# Autodesk Inventor assembly: Configuration 1
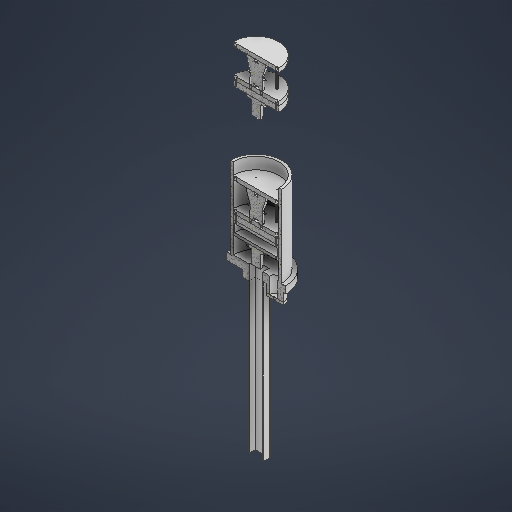
[picture p0: Inventor's stored thumbnail of the model, 512x512]
Saved by Autodesk Inventor 2025 (Build 290162000, 162)
## iProperties
Created: 2024-06-05
Part Number: Configuration 1
Document SubType Name: Assembly
Designer: AdminForWorker
Title: Printer Assembly v13
Author: AdminForWorker
## Documents named in this file (23)
- C:\Users\mayhe\OneDrive\Documents\GitHub\In-situ-monitoring-of-powder-bed-fusion-additive-manufacturing\system_development\Orichalcum\v0.2\Hardware_design\Full Printer Assembly\Printer Assembly.iam
- C:\Users\mayhe\OneDrive\Documents\GitHub\In-situ-monitoring-of-powder-bed-fusion-additive-manufacturing\system_development\Orichalcum\v0.2\Hardware_design\Full Printer Assembly\Printer Body v6.ipt
- C:\Users\mayhe\OneDrive\Documents\GitHub\In-situ-monitoring-of-powder-bed-fusion-additive-manufacturing\system_development\Orichalcum\v0.2\Hardware_design\Full Printer Assembly\Printer Frame.ipt
- C:\Users\mayhe\OneDrive\Documents\GitHub\In-situ-monitoring-of-powder-bed-fusion-additive-manufacturing\system_development\Orichalcum\v0.2\Hardware_design\Full Printer Assembly\overhead laser unit v1.ipt
- C:\Users\mayhe\OneDrive\Documents\GitHub\In-situ-monitoring-of-powder-bed-fusion-additive-manufacturing\system_development\Orichalcum\v0.2\Hardware_design\Full Printer Assembly\Part4.ipt
- C:\Users\mayhe\OneDrive\Documents\GitHub\In-situ-monitoring-of-powder-bed-fusion-additive-manufacturing\system_development\Orichalcum\v0.2\Hardware_design\custom-cover\cover\Updated Cover.ipt
- C:\Users\mayhe\OneDrive\Documents\GitHub\In-situ-monitoring-of-powder-bed-fusion-additive-manufacturing\system_development\Orichalcum\v0.2\Hardware_design\custom-cover\cylinder-parts\final-parts\Cylinder Bottom Ring.ipt
- C:\Users\mayhe\OneDrive\Documents\GitHub\In-situ-monitoring-of-powder-bed-fusion-additive-manufacturing\system_development\Orichalcum\v0.2\Hardware_design\custom-cover\cylinder-parts\final-parts\Cylinder Slidey Bit Housing.ipt
- C:\Users\mayhe\OneDrive\Documents\GitHub\In-situ-monitoring-of-powder-bed-fusion-additive-manufacturing\system_development\Orichalcum\v0.2\Hardware_design\custom-cover\cylinder-parts\Cylinder 80-20 Spacer_1.ipt
- C:\Users\mayhe\OneDrive\Documents\GitHub\In-situ-monitoring-of-powder-bed-fusion-additive-manufacturing\system_development\Orichalcum\v0.2\Hardware_design\custom-cover\cylinder-parts\Cylinder 80-20 Spacer_2.ipt
- C:\Users\mayhe\OneDrive\Documents\GitHub\In-situ-monitoring-of-powder-bed-fusion-additive-manufacturing\system_development\Orichalcum\v0.2\Hardware_design\custom-cover\8020-parts\20-2020-300.ipt
- C:\Users\mayhe\OneDrive\Documents\GitHub\In-situ-monitoring-of-powder-bed-fusion-additive-manufacturing\system_development\Orichalcum\v0.2\Hardware_design\custom-cover\cylinder-parts\cylinder-segments\Cylinder Segment .ipt
- C:\Users\mayhe\OneDrive\Documents\GitHub\In-situ-monitoring-of-powder-bed-fusion-additive-manufacturing\system_development\Orichalcum\v0.2\Hardware_design\custom-cover\cylinder-parts\final-parts\Cylinder Segment - 01.ipt
- C:\Users\mayhe\OneDrive\Documents\GitHub\In-situ-monitoring-of-powder-bed-fusion-additive-manufacturing\system_development\Orichalcum\v0.2\Hardware_design\custom-cover\cylinder-parts\final-parts\Cylinder Segment - Face.ipt
- C:\Users\mayhe\OneDrive\Documents\GitHub\In-situ-monitoring-of-powder-bed-fusion-additive-manufacturing\system_development\Orichalcum\v0.2\Hardware_design\custom-cover\cylinder-parts\final-parts\Cylinder Segment - 09.ipt
- C:\Users\mayhe\OneDrive\Documents\GitHub\In-situ-monitoring-of-powder-bed-fusion-additive-manufacturing\system_development\Orichalcum\v0.2\Hardware_design\custom-cover\cylinder-parts\final-parts\Cylinder Segment - 10.ipt
- C:\Users\mayhe\OneDrive\Documents\GitHub\In-situ-monitoring-of-powder-bed-fusion-additive-manufacturing\system_development\Orichalcum\v0.2\Hardware_design\custom-cover\cylinder-parts\cylinder-segments\Head Thing.ipt
- C:\Users\mayhe\OneDrive\Documents\GitHub\In-situ-monitoring-of-powder-bed-fusion-additive-manufacturing\system_development\Orichalcum\v0.2\Hardware_design\Full Printer Assembly\Plunger.ipt
- C:\Users\mayhe\OneDrive\Documents\GitHub\In-situ-monitoring-of-powder-bed-fusion-additive-manufacturing\system_development\Orichalcum\v0.2\Hardware_design\pzt-parts\PZT Assembly.iam
- C:\Users\mayhe\OneDrive\Documents\GitHub\In-situ-monitoring-of-powder-bed-fusion-additive-manufacturing\system_development\Orichalcum\v0.2\Hardware_design\Full Printer Assembly\Adapter Plate.ipt
- C:\Users\mayhe\OneDrive\Documents\GitHub\In-situ-monitoring-of-powder-bed-fusion-additive-manufacturing\system_development\Orichalcum\v0.2\Hardware_design\Full Printer Assembly\Build Plate.ipt
- C:\Users\mayhe\OneDrive\Documents\GitHub\In-situ-monitoring-of-powder-bed-fusion-additive-manufacturing\system_development\Orichalcum\v0.2\Hardware_design\Full Printer Assembly\Bottom Cap outlet.ipt
- C:\Users\mayhe\OneDrive\Documents\GitHub\In-situ-monitoring-of-powder-bed-fusion-additive-manufacturing\system_development\Orichalcum\v0.2\Hardware_design\pzt-parts\Capsule.ipt
## Components (28 placed, 21 different names)
1. Printer Frame:1 — Flush:1, Mate:1, Mate:2, Mate:3, Flush:2, Flush:3, Rotational:5, Rotational:6, Angle:3, Angle:4
2. Printer Body v6:1 — Flush:1, Mate:1, Mate:2, Mate:5, Mate:6, Mate:7, Angle:2
3. overhead laser unit v1:1 — Mate:4, Angle:1, Flush:4
4. Part4:1 — Mate:3, Flush:2, Flush:3, Mate:4, Angle:1, Flush:4
5. Plunger:1 — Rotational:6
6. Plunger:2 — Rotational:5, Cylindrical:1, Rotational:9, Mate:68, Angle:2, Cylindrical:2
7. Bottom Cap outlet:1 — Rotational:9, Mate:68
8. Updated Cover:1 — Mate:5, Mate:6, Mate:7, Rotational:4, Mate:53
9. Cylinder 80-20 Spacer_1:2 — Flush:5, Mate:29, Flush:6, Mate:30, Mate:59
10. Cylinder 80-20 Spacer_2:1 — Mate:26, Mate:60, Mate:61, Mate:62
11. Cylinder 80-20 Spacer_2:2 — Mate:47, Mate:54, Mate:55, Mate:56, Flush:7, Mate:57
12. Cylinder 80-20 Spacer_1:3 — Mate:64, Mate:65, Mate:66
13. 20-2020-300:1 — Mate:29, Flush:6, Mate:56, Flush:7, Mate:58
14. 20-2020-300:2 — Mate:26, Flush:5, Mate:52, Mate:63
15. Cylinder Segment - 01:1 — Mate:30, Mate:47, Rotational:2, Mate:48
16. Cylinder Slidey Bit Housing:1 — Rotational:2, Mate:48, Mate:50, Mate:51
17. Cylinder Segment - Face:2 — Rotational:3
18. Cylinder Segment - 09:3 — Mate:51, Mate:52
19. Cylinder Segment - 10:4 — Mate:50
20. Head Thing:1 — Rotational:3
21. Cylinder Bottom Ring:1 — Rotational:4, Mate:53, Mate:54, Mate:55, Mate:57, Mate:58, Mate:59, Mate:60, Mate:61, Mate:62, Mate:63, Mate:64, Mate:65, Mate:66
22. Build Plate:1 — Rotational:7, Rotational:8, Mate:67
23. Adapter Plate:1 — Rotational:7
24. PZT Assembly:1 [sub-assembly] — Rotational:8, Mate:67, Cylindrical:1, Angle:3
25. Capsule:1 — Rotational:10, Rotational:12, Mate:70
26. PZT Assembly:3 [sub-assembly] — Rotational:11, Cylindrical:2, Angle:4, Mate:69
27. Build Plate:3 — Rotational:10, Rotational:11, Mate:69, Mate:70
28. Adapter Plate:2 — Rotational:12
## Relationships (57: Mate 33, RevoluteJoint 11, Flush 7, Angle 4, CylindricalJoint 2)
- Flush:1: Printer Frame:1 ↔ Printer Body v6:1
- Mate:1: Printer Frame:1 ↔ Printer Body v6:1
- Mate:2 (92.5 mm): Printer Frame:1 ↔ Printer Body v6:1
- Mate:3: Printer Frame:1 ↔ Part4:1
- Flush:2 (28.5 mm): Printer Frame:1 ↔ Part4:1
- Flush:3 (-27 mm): Printer Frame:1 ↔ Part4:1
- Mate:4: overhead laser unit v1:1 ↔ Part4:1
- Angle:1 (179.9998 deg): overhead laser unit v1:1 ↔ Part4:1
- Flush:4 (-30 mm): overhead laser unit v1:1 ↔ Part4:1
- Mate:5: Printer Body v6:1 ↔ Updated Cover:1
- Mate:6: Printer Body v6:1 ↔ Updated Cover:1
- Mate:7: Printer Body v6:1 ↔ Updated Cover:1
- Mate:26: Cylinder 80-20 Spacer_2:1 ↔ 20-2020-300:2
- Flush:5: Cylinder 80-20 Spacer_1:2 ↔ 20-2020-300:2
- Mate:29: Cylinder 80-20 Spacer_1:2 ↔ 20-2020-300:1
- Flush:6: Cylinder 80-20 Spacer_1:2 ↔ 20-2020-300:1
- Mate:30: Cylinder 80-20 Spacer_1:2 ↔ Cylinder Segment - 01:1
- Mate:47: Cylinder 80-20 Spacer_2:2 ↔ Cylinder Segment - 01:1
- Rotational:2 [RevoluteJoint]: Cylinder Segment - 01:1 ↔ Cylinder Slidey Bit Housing:1
- Mate:48: Cylinder Segment - 01:1 ↔ Cylinder Slidey Bit Housing:1
- Mate:50: Cylinder Slidey Bit Housing:1 ↔ Cylinder Segment - 10:4
- Mate:51: Cylinder Slidey Bit Housing:1 ↔ Cylinder Segment - 09:3
- Mate:52: 20-2020-300:2 ↔ Cylinder Segment - 09:3
- Rotational:3 [RevoluteJoint]: Cylinder Segment - Face:2 ↔ Head Thing:1
- Rotational:4 [RevoluteJoint]: Updated Cover:1 ↔ Cylinder Bottom Ring:1
- Mate:53: Updated Cover:1 ↔ Cylinder Bottom Ring:1
- Mate:54: Cylinder 80-20 Spacer_2:2 ↔ Cylinder Bottom Ring:1
- Mate:55: Cylinder 80-20 Spacer_2:2 ↔ Cylinder Bottom Ring:1
- Mate:56: Cylinder 80-20 Spacer_2:2 ↔ 20-2020-300:1
- Flush:7: Cylinder 80-20 Spacer_2:2 ↔ 20-2020-300:1
- Mate:57: Cylinder 80-20 Spacer_2:2 ↔ Cylinder Bottom Ring:1
- Mate:58: 20-2020-300:1 ↔ Cylinder Bottom Ring:1
- Mate:59: Cylinder 80-20 Spacer_1:2 ↔ Cylinder Bottom Ring:1
- Mate:60: Cylinder 80-20 Spacer_2:1 ↔ Cylinder Bottom Ring:1
- Mate:61: Cylinder 80-20 Spacer_2:1 ↔ Cylinder Bottom Ring:1
- Mate:62: Cylinder 80-20 Spacer_2:1 ↔ Cylinder Bottom Ring:1
- Mate:63: 20-2020-300:2 ↔ Cylinder Bottom Ring:1
- Mate:64: Cylinder 80-20 Spacer_1:3 ↔ Cylinder Bottom Ring:1
- Mate:65: Cylinder 80-20 Spacer_1:3 ↔ Cylinder Bottom Ring:1
- Mate:66: Cylinder 80-20 Spacer_1:3 ↔ Cylinder Bottom Ring:1
- Rotational:5 [RevoluteJoint]: Printer Frame:1 ↔ Plunger:2
- Rotational:6 [RevoluteJoint]: Printer Frame:1 ↔ Plunger:1
- Rotational:7 [RevoluteJoint]: Build Plate:1 ↔ Adapter Plate:1
- Rotational:8 [RevoluteJoint]: Build Plate:1 ↔ PZT Assembly:1
- Mate:67: Build Plate:1 ↔ PZT Assembly:1
- Cylindrical:1: Plunger:2 ↔ PZT Assembly:1
- Rotational:9 [RevoluteJoint]: Plunger:2 ↔ Bottom Cap outlet:1
- Mate:68: Plunger:2 ↔ Bottom Cap outlet:1
- Angle:2 (0 deg): Printer Body v6:1 ↔ Plunger:2
- Angle:3 (0 deg): Printer Frame:1 ↔ PZT Assembly:1
- Rotational:10 [RevoluteJoint]: Capsule:1 ↔ Build Plate:3
- Rotational:11 [RevoluteJoint]: PZT Assembly:3 ↔ Build Plate:3
- Rotational:12 [RevoluteJoint]: Capsule:1 ↔ Adapter Plate:2
- Cylindrical:2: Plunger:2 ↔ PZT Assembly:3
- Angle:4 (0 deg): Printer Frame:1 ↔ PZT Assembly:3
- Mate:69: PZT Assembly:3 ↔ Build Plate:3
- Mate:70: Capsule:1 ↔ Build Plate:3
